# Autodesk Inventor assembly: 4x2 Angle
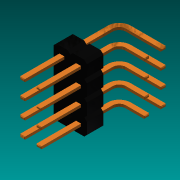
[picture p0: Inventor's stored thumbnail of the model, 180x180]
Saved by Autodesk Inventor 2015 (Build 190159000, 159)
## iProperties
Created: 2014-10-19
Part Number: 4x2 Angle
Document SubType Name: Assembly
Designer: Sawaiz Syed
Author: Sawaiz Syed
## Documents named in this file (2)
- C:\Users\Admin\SkyDrive\Classes\College\Semester 6\Research Project\Hardware\Transmitter 3D\Inventor\Radiation Dector\2.54 Breakaway\4x2 Angle.iam
- C:\Users\Admin\SkyDrive\Classes\College\Semester 6\Research Project\Hardware\Transmitter 3D\Inventor\Radiation Dector\2.54 Breakaway\1x2 Angle.iam
## Components (4 placed, 1 different names)
1. 1x2 Angle:1 [sub-assembly]
2. 1x2 Angle:2 [sub-assembly]
3. 1x2 Angle:3 [sub-assembly]
4. 1x2 Angle:4 [sub-assembly]
## Component patterns: (4 elements, first: 1x2 Angle:1)
